# Autodesk Inventor assembly: mabuchi 555+IG32
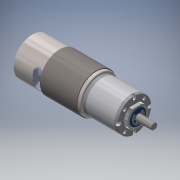
[picture p0: Inventor's stored thumbnail of the model, 180x180]
Saved by Autodesk Inventor 2019 (Build 230136000, 136)
## iProperties
Created: 2018-10-18
Part Number: mabuchi 555+IG32
Material: 一般
Document SubType Name: Assembly
Designer: shun
Author: shun
## Documents named in this file (3)
- C:\Users\shun\Documents\Inventor\MR2\ヘッケン2\mabuchi 555+IG32.iam
- C:\Users\shun\Documents\Inventor\MR2\ヘッケン2\Mabuchi 555.ipt
- C:\Users\shun\Documents\Inventor\MR2\ヘッケン2\IG-32_51以上.ipt
## Components (2 placed, 2 different names)
1. Mabuchi 555:1 — メイト:1, メイト:2, 角度:1
2. IG-32_51以上:1 — メイト:1, メイト:2, 角度:1
## Relationships (3: Mate 2, Angle 1)
- メイト:1 [Mate]: Mabuchi 555:1 ↔ IG-32_51以上:1
- メイト:2 [Mate]: Mabuchi 555:1 ↔ IG-32_51以上:1
- 角度:1 [Angle] (0 deg): Mabuchi 555:1 ↔ IG-32_51以上:1
